# Autodesk Inventor assembly: Assembly
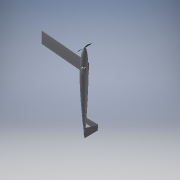
[picture p0: Inventor's stored thumbnail of the model, 180x180]
Saved by Autodesk Inventor 2019 (Build 230136000, 136)
## iProperties
Created: 2019-04-06
Part Number: Assembly
Document SubType Name: Assembly
Designer: albaa
Mass: 1701.42 g
Surface Area: 26127.2 cm^2
Volume: 7650.91 cm^3
Density: 0.222382 g/cm^3
Author: albaa
## Documents named in this file (9)
- C:\Users\albaa\Google Drive\McGill OneDrive\McGill\Courses\13_WINTER 2019\MECH 532\Project\REPO_mech532-project\CAD\Assembly.iam
- C:\Users\albaa\Google Drive\McGill OneDrive\McGill\Courses\13_WINTER 2019\MECH 532\Project\REPO_mech532-project\CAD\hTail_wing.ipt
- C:\Users\albaa\Google Drive\McGill OneDrive\McGill\Courses\13_WINTER 2019\MECH 532\Project\REPO_mech532-project\CAD\main_wing.ipt
- C:\Users\albaa\Google Drive\McGill OneDrive\McGill\Courses\13_WINTER 2019\MECH 532\Project\REPO_mech532-project\CAD\vTail_wing.ipt
- C:\Users\albaa\Google Drive\McGill OneDrive\McGill\Courses\13_WINTER 2019\MECH 532\Project\REPO_mech532-project\CAD\motor.ipt
- C:\Users\albaa\Google Drive\McGill OneDrive\McGill\Courses\13_WINTER 2019\MECH 532\Project\REPO_mech532-project\CAD\propeller.ipt
- C:\Users\albaa\Google Drive\McGill OneDrive\McGill\Courses\13_WINTER 2019\MECH 532\Project\REPO_mech532-project\CAD\battery.ipt
- C:\Users\albaa\Google Drive\McGill OneDrive\McGill\Courses\13_WINTER 2019\MECH 532\Project\REPO_mech532-project\CAD\payload.ipt
- C:\Users\albaa\Google Drive\McGill OneDrive\McGill\Courses\13_WINTER 2019\MECH 532\Project\REPO_mech532-project\CAD\fuselage_2.ipt
## Components (8 placed, 8 different names)
1. fuselage_2:1 — Flush:14
2. hTail_wing:1 — Flush:5, Flush:6
3. main_wing:1 — Mate:3, Flush:11
4. vTail_wing:1 — Flush:8, Flush:14
5. motor:1 — Mate:5, Mate:6
6. propeller:1 — Mate:5, Mate:6
7. battery:1
8. payload:1
## Relationships (17: Flush 11, Mate 6)
- [Flush]: fuselage_2:1
- [Flush]: fuselage_2:1
- [Mate] (-500 mm): fuselage_2:1 ↔ main_wing:1
- Flush:5: hTail_wing:1
- Flush:6 (-250 mm): hTail_wing:1
- [Mate] (-1400 mm): fuselage_2:1 ↔ hTail_wing:1
- [Flush]: fuselage_2:1 ↔ vTail_wing:1
- Flush:8: vTail_wing:1
- [Flush]: fuselage_2:1
- Mate:3 (70 mm): main_wing:1
- Flush:11: main_wing:1
- [Mate]: fuselage_2:1 ↔ motor:1
- Mate:5: motor:1 ↔ propeller:1
- Mate:6: motor:1 ↔ propeller:1
- [Flush]: fuselage_2:1 ↔ battery:1
- [Flush]: fuselage_2:1 ↔ payload:1
- Flush:14 (-1340 mm): fuselage_2:1 ↔ vTail_wing:1
